# Autodesk Inventor assembly: 4 Wire - Pivot Action
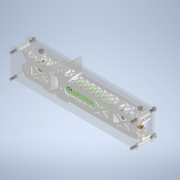
[picture p0: Inventor's stored thumbnail of the model, 180x180]
Saved by Autodesk Inventor 2021 (Build 250183000, 183)
## iProperties
Created: 2020-06-16
Part Number: 4 Wire - Pivot Action
Document SubType Name: Assembly
Designer: lucas
Project: 4Wire-FDM
Author: lucas
Revision Number: RLS_004
## Documents named in this file (9)
- C:\Users\lucas\Nextcloud\HackerSpace\HV Home Battery Storage Project\Concepts & Storyboards\18650 4wire Holder\Araknid-4Wire-FDM-Slot-x1.iam
- C:\Users\lucas\Nextcloud\HackerSpace\HV Home Battery Storage Project\Concepts & Storyboards\18650 4wire Holder\Shared Parts\18650-VTC4.ipt
- C:\Users\lucas\Nextcloud\HackerSpace\HV Home Battery Storage Project\Concepts & Storyboards\18650 4wire Holder\4Wire-FDM-Slot\Template-Fixture-Mid.ipt
- C:\Users\lucas\Nextcloud\HackerSpace\HV Home Battery Storage Project\Concepts & Storyboards\18650 4wire Holder\4Wire-FDM-Slot\Template-Fixture-Top.ipt
- C:\Users\lucas\Nextcloud\HackerSpace\HV Home Battery Storage Project\Concepts & Storyboards\18650 4wire Holder\4Wire-FDM-Slot\Template-Fixture-Bottom.ipt
- C:\Users\lucas\Nextcloud\HackerSpace\HV Home Battery Storage Project\Concepts & Storyboards\18650 4wire Holder\Shared Parts\Standoff-Threaded-M3x18mm.ipt
- C:\Users\lucas\Documents\Inventor\Content Center Files\R2021\en-US\U 2605\Unbrako - M3 x  20(5).ipt
- C:\Users\lucas\Nextcloud\HackerSpace\HV Home Battery Storage Project\Concepts & Storyboards\18650 4wire Holder\4Wire-FDM-Slot\4Wire-FDM-Slot.iam
- C:\Users\lucas\Nextcloud\HackerSpace\HV Home Battery Storage Project\Concepts & Storyboards\18650 4wire Holder\4Wire-FDM-Slot\4Wire-FDM-Pivot.iam
## Components (14 placed, 8 different names)
1. 18650-VTC4:1 — Mate:12
2. Template-Fixture-Mid:1 — Mate:1, Flush:1, Flush:2, Mate:11, Flush:4, Flush:5, Rotational:4, Rotational:5
3. Template-Fixture-Top:1 — Mate:1, Flush:1, Flush:2, Insert:1, Insert:2, Insert:3, Insert:4
4. Template-Fixture-Bottom:1 — Mate:11, Flush:4, Flush:5, Rotational:1, Rigid:1, Rotational:2, Rotational:3
5. Standoff-TH-M3x18mm:1 — Rotational:1
6. Standoff-TH-M3x18mm:2 — Rigid:1
7. Standoff-TH-M3x18mm:3 — Rotational:3
8. Standoff-TH-M3x18mm:4 — Rotational:2
9. Unbrako Hex Socket Button Cap - Metric M3 x 20:1 — Insert:1
10. Unbrako Hex Socket Button Cap - Metric M3 x 20:2 — Insert:2
11. Unbrako Hex Socket Button Cap - Metric M3 x 20:3 — Insert:3
12. Unbrako Hex Socket Button Cap - Metric M3 x 20:4 — Insert:4
13. 4Wire-FDM-Slot:1 [sub-assembly] — Rotational:4, Rotation:1, Mate:12
14. 4Wire-FDM-Pivot:1 [sub-assembly] — Rotational:5, Rotation:1
## Relationships (18: RevoluteJoint 5, Flush 4, Insert 4, Mate 3, WeldJoint 1, RelateRotation 1)
- Mate:1: Template-Fixture-Mid:1 ↔ Template-Fixture-Top:1
- Flush:1: Template-Fixture-Mid:1 ↔ Template-Fixture-Top:1
- Flush:2: Template-Fixture-Mid:1 ↔ Template-Fixture-Top:1
- Mate:11 (18 mm): Template-Fixture-Mid:1 ↔ Template-Fixture-Bottom:1
- Flush:4: Template-Fixture-Mid:1 ↔ Template-Fixture-Bottom:1
- Flush:5: Template-Fixture-Mid:1 ↔ Template-Fixture-Bottom:1
- Rotational:1 [RevoluteJoint]: Template-Fixture-Bottom:1 ↔ Standoff-TH-M3x18mm:1
- Rigid:1 [WeldJoint]: Template-Fixture-Bottom:1 ↔ Standoff-TH-M3x18mm:2
- Rotational:2 [RevoluteJoint]: Template-Fixture-Bottom:1 ↔ Standoff-TH-M3x18mm:4
- Rotational:3 [RevoluteJoint]: Template-Fixture-Bottom:1 ↔ Standoff-TH-M3x18mm:3
- Insert:1: Template-Fixture-Top:1 ↔ Unbrako Hex Socket Button Cap - Metric M3 x 20:1
- Insert:2: Template-Fixture-Top:1 ↔ Unbrako Hex Socket Button Cap - Metric M3 x 20:2
- Insert:3: Template-Fixture-Top:1 ↔ Unbrako Hex Socket Button Cap - Metric M3 x 20:3
- Insert:4: Template-Fixture-Top:1 ↔ Unbrako Hex Socket Button Cap - Metric M3 x 20:4
- Rotational:4 [RevoluteJoint] (3.25 mm): Template-Fixture-Mid:1 ↔ 4Wire-FDM-Slot:1
- Rotational:5 [RevoluteJoint] (3.25 mm): Template-Fixture-Mid:1 ↔ 4Wire-FDM-Pivot:1
- Rotation:1 [RelateRotation] (2.5533 ul): 4Wire-FDM-Slot:1 ↔ 4Wire-FDM-Pivot:1
- Mate:12: 18650-VTC4:1 ↔ 4Wire-FDM-Slot:1
